# Autodesk Inventor assembly: SACMI PH1500 FEEDER FRAME
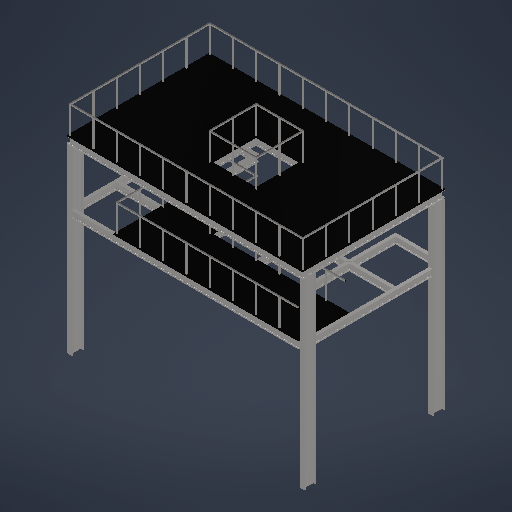
[picture p0: Inventor's stored thumbnail of the model, 512x512]
Saved by Autodesk Inventor 2025 (Build 290162000, 162)
## iProperties
Created: 2024-05-05
Part Number: SACMI PH1500 FEEDER FRAME
Document SubType Name: Assembly
Designer: zulet
Author: zulet
## Documents named in this file (83)
- D:\UNAL\2024-1S\APM\Digital Factory\SACMI PH1500\Frame\SACMI PH1500 FEEDER FRAME.iam
- D:\UNAL\2024-1S\APM\Digital Factory\SACMI PH1500\Frame\FEEDER SKELETON.ipt
- D:\UNAL\2024-1S\APM\Digital Factory\SACMI PH1500\Frame\DIN 1025 IPE 360 1714952337686.ipt
- D:\UNAL\2024-1S\APM\Digital Factory\SACMI PH1500\Frame\DIN 1025 IPE 360 1714952337738.ipt
- D:\UNAL\2024-1S\APM\Digital Factory\SACMI PH1500\Frame\DIN 1025 IPE 360 1714952337789.ipt
- D:\UNAL\2024-1S\APM\Digital Factory\SACMI PH1500\Frame\DIN 1025 IPE 360 1714952337840.ipt
- D:\UNAL\2024-1S\APM\Digital Factory\SACMI PH1500\Frame\DIN 1025 IPE 360 1714952338238.ipt
- D:\UNAL\2024-1S\APM\Digital Factory\SACMI PH1500\Frame\DIN 1025 IPE 360 1714952339458.ipt
- D:\UNAL\2024-1S\APM\Digital Factory\SACMI PH1500\Frame\DIN 1025 IPE 360 1714952339502.ipt
- D:\UNAL\2024-1S\APM\Digital Factory\SACMI PH1500\Frame\DIN 1025 IPE 360 1714952339545.ipt
- D:\UNAL\2024-1S\APM\Digital Factory\SACMI PH1500\Frame\DIN 1025 IPE 220 1714954189621.ipt
- D:\UNAL\2024-1S\APM\Digital Factory\SACMI PH1500\Frame\DIN 1025 IPE 220 1714954189674.ipt
- D:\UNAL\2024-1S\APM\Digital Factory\SACMI PH1500\Frame\DIN 1025 IPE 220 1714954189725.ipt
- D:\UNAL\2024-1S\APM\Digital Factory\SACMI PH1500\Frame\DIN 1025 IPE 220 1714954189777.ipt
- D:\UNAL\2024-1S\APM\Digital Factory\SACMI PH1500\Frame\DIN 1025 IPE 220 1714954189830.ipt
- D:\UNAL\2024-1S\APM\Digital Factory\SACMI PH1500\Frame\DIN 1025 IPE 220 1714954189880.ipt
- D:\UNAL\2024-1S\APM\Digital Factory\SACMI PH1500\Frame\DIN 1025 IPE 220 1714954189928.ipt
- D:\UNAL\2024-1S\APM\Digital Factory\SACMI PH1500\Frame\DIN 1025 IPE 220 1714954189976.ipt
- D:\UNAL\2024-1S\APM\Digital Factory\SACMI PH1500\Frame\DIN 1025 IPE 220 1714954190025.ipt
- D:\UNAL\2024-1S\APM\Digital Factory\SACMI PH1500\Frame\DIN 1025 IPE 220 1714954190075.ipt
- D:\UNAL\2024-1S\APM\Digital Factory\SACMI PH1500\Frame\DIN 1025 IPE 220 1714954190126.ipt
- D:\UNAL\2024-1S\APM\Digital Factory\SACMI PH1500\Frame\DIN 1025 IPE 220 1714954190175.ipt
- D:\UNAL\2024-1S\APM\Digital Factory\SACMI PH1500\Frame\DIN 1025 IPE 220 1714954190225.ipt
- D:\UNAL\2024-1S\APM\Digital Factory\SACMI PH1500\Frame\DIN 1025 IPE 220 1714954190275.ipt
- D:\UNAL\2024-1S\APM\Digital Factory\SACMI PH1500\Frame\DIN 1025 IPE 220 1714954190323.ipt
- D:\UNAL\2024-1S\APM\Digital Factory\SACMI PH1500\Frame\DIN 1025 IPE 220 1714954190374.ipt
- D:\UNAL\2024-1S\APM\Digital Factory\SACMI PH1500\Frame\DIN 1025 IPE 220 1714954190424.ipt
- D:\UNAL\2024-1S\APM\Digital Factory\SACMI PH1500\Frame\DIN 1025 IPE 220 1714954190474.ipt
- D:\UNAL\2024-1S\APM\Digital Factory\SACMI PH1500\Frame\DIN 1025 IPE 220 1714954190523.ipt
- D:\UNAL\2024-1S\APM\Digital Factory\SACMI PH1500\Frame\DIN 1025 IPE 220 1714954190574.ipt
- D:\UNAL\2024-1S\APM\Digital Factory\SACMI PH1500\Frame\DIN 1025 IPE 220 1714954190622.ipt
- D:\UNAL\2024-1S\APM\Digital Factory\SACMI PH1500\Frame\DIN 1025 IPE 220 1714954190672.ipt
- D:\UNAL\2024-1S\APM\Digital Factory\SACMI PH1500\Frame\DIN 1025 IPE 220 1714954190723.ipt
- D:\UNAL\2024-1S\APM\Digital Factory\SACMI PH1500\Frame\DIN 1025 IPE 220 1714954190772.ipt
- D:\UNAL\2024-1S\APM\Digital Factory\SACMI PH1500\Frame\DIN 1025 IPE 220 1714954190825.ipt
- D:\UNAL\2024-1S\APM\Digital Factory\SACMI PH1500\Frame\DIN 1025 IPE 220 1714954190876.ipt
- D:\UNAL\2024-1S\APM\Digital Factory\SACMI PH1500\Frame\DIN 1025 IPE 220 1714954190924.ipt
- D:\UNAL\2024-1S\APM\Digital Factory\SACMI PH1500\Frame\DIN 1025 IPE 220 1714954190974.ipt
- D:\UNAL\2024-1S\APM\Digital Factory\SACMI PH1500\Frame\DIN 1025 IPE 220 1714954191023.ipt
- D:\UNAL\2024-1S\APM\Digital Factory\SACMI PH1500\Frame\DIN 1025 IPE 220 1714954191079.ipt
- D:\UNAL\2024-1S\APM\Digital Factory\SACMI PH1500\Frame\DIN 1025 IPE 220 1714954191128.ipt
- D:\UNAL\2024-1S\APM\Digital Factory\SACMI PH1500\Frame\DIN 1025 IPE 220 1714954191177.ipt
- D:\UNAL\2024-1S\APM\Digital Factory\SACMI PH1500\Frame\DIN 1025 IPE 220 1714954191227.ipt
- D:\UNAL\2024-1S\APM\Digital Factory\SACMI PH1500\Frame\DIN 1025 IPE 220 1714954191276.ipt
- D:\UNAL\2024-1S\APM\Digital Factory\SACMI PH1500\Frame\DIN 1025 IPE 220 1714954191325.ipt
- D:\UNAL\2024-1S\APM\Digital Factory\SACMI PH1500\Frame\DIN 1025 IPE 220 1714954191377.ipt
- D:\UNAL\2024-1S\APM\Digital Factory\SACMI PH1500\Frame\DIN 1025 IPE 220 1714954191425.ipt
- D:\UNAL\2024-1S\APM\Digital Factory\SACMI PH1500\Frame\DIN 1025 IPE 220 1714954191476.ipt
- D:\UNAL\2024-1S\APM\Digital Factory\SACMI PH1500\Frame\DIN 1025 IPE 220 1714954191526.ipt
- D:\UNAL\2024-1S\APM\Digital Factory\SACMI PH1500\Frame\DIN 1025 IPE 220 1714954191574.ipt
- D:\UNAL\2024-1S\APM\Digital Factory\SACMI PH1500\Frame\DIN 1025 IPE 220 1714954191623.ipt
- D:\UNAL\2024-1S\APM\Digital Factory\SACMI PH1500\Frame\DIN 1025 IPE 220 1714954191672.ipt
- D:\UNAL\2024-1S\APM\Digital Factory\SACMI PH1500\Frame\DIN 1025 IPE 220 1714954191722.ipt
- D:\UNAL\2024-1S\APM\Digital Factory\SACMI PH1500\Frame\DIN 1025 IPE 220 1714954191779.ipt
- D:\UNAL\2024-1S\APM\Digital Factory\SACMI PH1500\Frame\DIN 1025 IPE 220 1714954191832.ipt
- D:\UNAL\2024-1S\APM\Digital Factory\SACMI PH1500\Frame\DIN 1025 IPE 220 1714954191882.ipt
- D:\UNAL\2024-1S\APM\Digital Factory\SACMI PH1500\Frame\DIN 1025 IPE 220 1714954191932.ipt
- D:\UNAL\2024-1S\APM\Digital Factory\SACMI PH1500\Frame\DIN 1025 IPE 220 1714954191982.ipt
- D:\UNAL\2024-1S\APM\Digital Factory\SACMI PH1500\Frame\DIN 1025 IPE 220 1714954192031.ipt
- D:\UNAL\2024-1S\APM\Digital Factory\SACMI PH1500\Frame\DIN 1025 IPE 220 1714954192082.ipt
- D:\UNAL\2024-1S\APM\Digital Factory\SACMI PH1500\Frame\DIN 1025 IPE 220 1714954192132.ipt
- D:\UNAL\2024-1S\APM\Digital Factory\SACMI PH1500\Frame\DIN 1025 IPE 220 1714954192191.ipt
- D:\UNAL\2024-1S\APM\Digital Factory\SACMI PH1500\Frame\DIN 1025 IPE 220 1714954192240.ipt
- D:\UNAL\2024-1S\APM\Digital Factory\SACMI PH1500\Frame\DIN 1025 IPE 220 1714954192290.ipt
- D:\UNAL\2024-1S\APM\Digital Factory\SACMI PH1500\Frame\DIN 1025 IPE 220 1714954192338.ipt
- D:\UNAL\2024-1S\APM\Digital Factory\SACMI PH1500\Frame\DIN 1025 IPE 220 1714954192389.ipt
- D:\UNAL\2024-1S\APM\Digital Factory\SACMI PH1500\Frame\DIN 1025 IPE 220 1714954192438.ipt
- D:\UNAL\2024-1S\APM\Digital Factory\SACMI PH1500\Frame\DIN 1025 IPE 220 1714954192486.ipt
- D:\UNAL\2024-1S\APM\Digital Factory\SACMI PH1500\Frame\DIN 1025 IPE 220 1714954192540.ipt
- D:\UNAL\2024-1S\APM\Digital Factory\SACMI PH1500\Frame\DIN 1025 IPE 220 1714954192589.ipt
- D:\UNAL\2024-1S\APM\Digital Factory\SACMI PH1500\Frame\DIN 1025 IPE 220 1714954192637.ipt
- D:\UNAL\2024-1S\APM\Digital Factory\SACMI PH1500\Frame\DIN 1025 IPE 220 1714954192685.ipt
- D:\UNAL\2024-1S\APM\Digital Factory\SACMI PH1500\Frame\DIN 1025 IPE 220 1714954192734.ipt
- D:\UNAL\2024-1S\APM\Digital Factory\SACMI PH1500\Frame\DIN 1025 IPE 220 1714954192783.ipt
- D:\UNAL\2024-1S\APM\Digital Factory\SACMI PH1500\Frame\DIN 1025 IPE 220 1714954192835.ipt
- D:\UNAL\2024-1S\APM\Digital Factory\SACMI PH1500\Frame\DIN 1025 IPE 220 1714954192898.ipt
- D:\UNAL\2024-1S\APM\Digital Factory\SACMI PH1500\Frame\DIN 1025 IPE 220 1714954192963.ipt
- D:\UNAL\2024-1S\APM\Digital Factory\SACMI PH1500\Frame\DIN 1025 IPE 220 1714954193028.ipt
- D:\UNAL\2024-1S\APM\Digital Factory\SACMI PH1500\Frame\DIN 1025 IPE 220 1714954193094.ipt
- D:\UNAL\2024-1S\APM\Digital Factory\SACMI PH1500\Frame\DIN 1025 IPE 220 1714954193162.ipt
- D:\UNAL\2024-1S\APM\Digital Factory\SACMI PH1500\Frame\DIN 1025 IPE 220 1714954193230.ipt
- D:\UNAL\2024-1S\APM\Digital Factory\SACMI PH1500\SecondFloor.ipt
- D:\UNAL\2024-1S\APM\Digital Factory\SACMI PH1500\FirstFloorP.ipt
## Components (82 placed, 12 different names)
1. Reference Skeleton
2. DIN 1025 IPE 220 - 1555:1
3. DIN 1025 IPE 220 - 1497,05:1
4. DIN 1025 IPE 220 - 1555:2
5. DIN 1025 IPE 220 - 1497,05:1
6. DIN 1025 IPE 220 - 1500:3
7. DIN 1025 IPE 220 - 1555:4
8. DIN 1025 IPE 220 - 1497,05:1
9. DIN 1025 IPE 220 - 1555:5
10. DIN 1025 IPE 220 - 1497,05:1
11. DIN 1025 IPE 220 - 1500:6
12. DIN 1025 IPE 220 - 1500:7
13. DIN 1025 IPE 220 - 1497,05:1
14. DIN 1025 IPE 220 - 1500:8
15. DIN 1025 IPE 220 - 1500:9
16. DIN 1025 IPE 220 - 1500:10
17. DIN 1025 IPE 220 - 1500:11
18. DIN 1025 IPE 220 - 1500:12
19. DIN 1025 IPE 220 - 1497,05:1
20. DIN 1025 IPE 220 - 1500:13
21. DIN 1025 IPE 220 - 1500:14
22. DIN 1025 IPE 220 - 1500:15
23. DIN 1025 IPE 220 - 1497,05:1
24. DIN 1025 IPE 220 - 1500:16
25. DIN 1025 IPE 220 - 1497,05:1
26. DIN 1025 IPE 220 - 1500:17
27. DIN 1025 IPE 220 - 1500:18
28. DIN 1025 IPE 220 - 1497,05:1
29. DIN 1025 IPE 220 - 1555:19
30. DIN 1025 IPE 220 - 1555:20
31. DIN 1025 IPE 220 - 1497,05:1
32. DIN 1025 IPE 220 - 1500:21
33. DIN 1025 IPE 220 - 1500:22
34. DIN 1025 IPE 220 - 1500:23
35. DIN 1025 IPE 220 - 1497,05:1
36. DIN 1025 IPE 220 - 1497,05:1
37. DIN 1025 IPE 220 - 1555:22
38. DIN 1025 IPE 220 - 1555:23 — Flush:1
39. DIN 1025 IPE 220 - 1500:24
40. DIN 1025 IPE 360 - 1890:1
41. DIN 1025 IPE 360 - 1890:2
42. DIN 1025 IPE 360 - 1890:3
43. DIN 1025 IPE 360 - 1890:4
44. DIN 1025 IPE 220 - 1470:1
45. DIN 1025 IPE 220 - 1555:2
46. DIN 1025 IPE 220 - 1140:25
47. DIN 1025 IPE 220 - 1497,05:26
48. DIN 1025 IPE 220 - 1500:27
49. DIN 1025 IPE 220 - 1500:28
50. DIN 1025 IPE 220 - 1470:1
51. DIN 1025 IPE 360 - 4000:5
52. DIN 1025 IPE 220 - 1140:29
53. DIN 1025 IPE 220 - 1555:2
54. DIN 1025 IPE 220 - 1497,05:30
55. DIN 1025 IPE 220 - 1500:31
56. DIN 1025 IPE 220 - 1497,05:32
57. DIN 1025 IPE 220 - 1500:33
58. DIN 1025 IPE 220 - 1555:1
59. DIN 1025 IPE 220 - 1610:1
60. DIN 1025 IPE 220 - 1555:2
61. DIN 1025 IPE 220 - 1500:32
62. DIN 1025 IPE 220 - 1500:33
63. DIN 1025 IPE 220 - 1500:34
64. DIN 1025 IPE 220 - 1500:35
65. DIN 1025 IPE 220 - 1500:36
66. DIN 1025 IPE 220 - 1497,05:37
67. DIN 1025 IPE 220 - 1497,05:38
68. DIN 1025 IPE 220 - 1140:39
69. DIN 1025 IPE 220 - 1415:40
70. DIN 1025 IPE 220 - 1500:41
71. DIN 1025 IPE 220 - 1497,05:42
72. DIN 1025 IPE 220 - 1500:43
73. DIN 1025 IPE 220 - 1497,05:44
74. DIN 1025 IPE 220 - 1500:45
75. DIN 1025 IPE 220 - 1497,05:46
76. DIN 1025 IPE 220 - 1415:47
77. DIN 1025 IPE 220 - 1140:48 — Flush:2
78. DIN 1025 IPE 360 - 4000:6
79. DIN 1025 IPE 360 - 4000:7
80. DIN 1025 IPE 360 - 4000:8
81. SecondFloor:1 — Flush:1
82. FirstFloorP:1 — Flush:2
## Relationships (2: Flush 2)
- Flush:1: DIN 1025 IPE 220 - 1555:23 ↔ SecondFloor:1
- Flush:2: DIN 1025 IPE 220 - 1140:48 ↔ FirstFloorP:1
